# Autodesk Inventor assembly: Tail
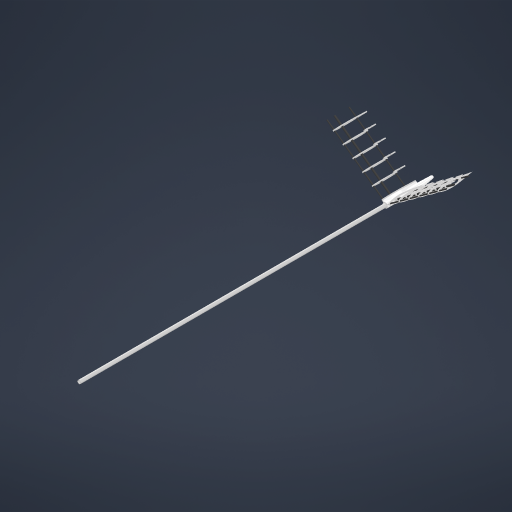
[picture p0: Inventor's stored thumbnail of the model, 512x512]
Saved by Autodesk Inventor 2023 (Build 270158000, 158)
## iProperties
Created: 2023-01-05
Part Number: Tail
Document SubType Name: Assembly
Designer: szykr
Author: szykr
## Documents named in this file (7)
- D:\Folder Instalacyjny\GitHub Pliki\Solaris\new model\Tail\Tail.iam
- D:\Folder Instalacyjny\GitHub Pliki\Solaris\new model\wingspar.ipt
- D:\Folder Instalacyjny\GitHub Pliki\Solaris\new model\Tail\Tżebro default.ipt
- D:\Folder Instalacyjny\GitHub Pliki\Solaris\new model\Tail\Twingspar.ipt
- D:\Folder Instalacyjny\GitHub Pliki\Solaris\new model\Tail\TsmallSpar.ipt
- D:\Folder Instalacyjny\GitHub Pliki\Solaris\new model\Tail\Zebro_z_lotka.iam
- D:\Folder Instalacyjny\GitHub Pliki\Solaris\new model\Tail\Tmouint-edito.ipt
## Components (22 placed, 6 different names)
1. wingspar:1 — Insert:1
2. Tżebro default:1
3. Tżebro default:2
4. Twingspar:1 — Insert:6, Mate:1, Mate:10, Mate:12
5. Twingspar:2 — Insert:3, Mate:4, Mate:7, Mate:9
6. TsmallSpar:1 — Insert:4
7. TsmallSpar:2 — Insert:2, Mate:5
8. TsmallSpar:3 — Insert:7
9. TsmallSpar:4 — Insert:5, Mate:2
10. Tżebro default:3 — Mate:9, Flush:1
11. Tżebro default:4 — Mate:12, Flush:2
12. Tmouint-edito:1 — Insert:1, Insert:2, Insert:3, Insert:4, Insert:5, Insert:6, Insert:7, Mate:3, Mate:6, Mate:8, Mate:11
13. Tżebro default:5 — Mate:1, Mate:2, Mate:3
14. Tżebro default:6 — Mate:4, Mate:5, Mate:6
15. Zebro_z_lotka:1 [sub-assembly] — Mate:10, Mate:11
16. Zebro_z_lotka:3 [sub-assembly]
17. Zebro_z_lotka:4 [sub-assembly]
18. Zebro_z_lotka:5 [sub-assembly] — Flush:2
19. Zebro_z_lotka:2 [sub-assembly] — Mate:7, Mate:8
20. Zebro_z_lotka:6 [sub-assembly]
21. Zebro_z_lotka:7 [sub-assembly]
22. Zebro_z_lotka:8 [sub-assembly] — Flush:1
## Component patterns: (4 elements, first: Zebro_z_lotka:1), (4 elements, first: Zebro_z_lotka:2)
## Relationships (21: Mate 12, Insert 7, Flush 2)
- Insert:1: wingspar:1 ↔ Tmouint-edito:1
- Insert:2 (-4.366 mm): TsmallSpar:2 ↔ Tmouint-edito:1
- Insert:3 (-4.366 mm): Twingspar:2 ↔ Tmouint-edito:1
- Insert:4 (-4.366 mm): TsmallSpar:1 ↔ Tmouint-edito:1
- Insert:5 (-4.366 mm): TsmallSpar:4 ↔ Tmouint-edito:1
- Insert:6 (-4.366 mm): Twingspar:1 ↔ Tmouint-edito:1
- Insert:7 (-4.366 mm): TsmallSpar:3 ↔ Tmouint-edito:1
- Mate:1: Twingspar:1 ↔ Tżebro default:5
- Mate:2: TsmallSpar:4 ↔ Tżebro default:5
- Mate:3: Tmouint-edito:1 ↔ Tżebro default:5
- Mate:4: Twingspar:2 ↔ Tżebro default:6
- Mate:5: TsmallSpar:2 ↔ Tżebro default:6
- Mate:6: Tmouint-edito:1 ↔ Tżebro default:6
- Mate:7: Twingspar:2 ↔ Zebro_z_lotka:2
- Mate:8 (35.5 mm): Tmouint-edito:1 ↔ Zebro_z_lotka:2
- Mate:9: Twingspar:2 ↔ Tżebro default:3
- Flush:1 (35.5 mm): Tżebro default:3 ↔ Zebro_z_lotka:8
- Mate:10: Twingspar:1 ↔ Zebro_z_lotka:1
- Mate:11 (35.5 mm): Tmouint-edito:1 ↔ Zebro_z_lotka:1
- Mate:12: Twingspar:1 ↔ Tżebro default:4
- Flush:2 (35.5 mm): Tżebro default:4 ↔ Zebro_z_lotka:5
## Named parameters: dlugosc = 213 mm, lotki = 4, ilosc_zeber = 6, spacing = 35.5 mm
